# Autodesk Inventor assembly: Lady Brown LS Axle (Left)
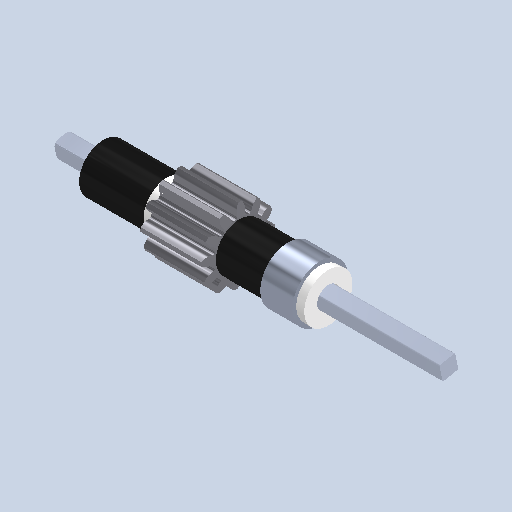
[picture p0: Inventor's stored thumbnail of the model, 512x512]
Saved by Autodesk Inventor 2025.1 (Build 291241020, 241B)
## iProperties
Created: 2024-12-19
Part Number: Lady Brown LS Axle (Left)
Document SubType Name: Assembly
Designer: Juan
Author: Juan
## Documents named in this file (11)
- C:\Users\AtuStem\Documents\GitHub\ATUM-V5RC-High-Stakes-CAD\Robot\Subassemblies\Lady Brown LS Axle (Left).iam
- C:\Users\AtuStem\Documents\GitHub\ATUM-V5RC-High-Stakes-CAD\VEX-CAD-Inventor\Motion\Shaft LS\Shaft LS\Shaft LS 3.0.ipt
- C:\Users\Juan\Documents\GitHub\ATUM-VRC-High-Stakes-CAD\VEX-CAD-Inventor\Motion\Shaft LS\Shaft LS.ipt
- C:\Users\AtuStem\Documents\GitHub\ATUM-V5RC-High-Stakes-CAD\VEX-CAD-Inventor\Motion\Shaft LS\Shaft Collar Metal\Shaft Collar No Screw.ipt
- C:\Users\AtuStem\Documents\GitHub\ATUM-V5RC-High-Stakes-CAD\VEX-CAD-Inventor\Motion\Gears\HS Gear\HS 12T Gear, Square.iam
- C:\Users\Juan\Documents\GitHub\ATUM-VRC-High-Stakes-CAD\VEX-CAD-Inventor\Motion\Gears\HS Gear.iam
- C:\Users\AtuStem\Documents\GitHub\ATUM-V5RC-High-Stakes-CAD\VEX-CAD-Inventor\Motion\Spacers\Spacer Nylon .375 OD\NSpacer .375 OD x .375.ipt
- C:\Users\Juan\Documents\GitHub\ATUM-VRC-High-Stakes-CAD\VEX-CAD-Inventor\Motion\Spacers\Spacer Nylon .375 OD.ipt
- C:\Users\AtuStem\Documents\GitHub\ATUM-V5RC-High-Stakes-CAD\VEX-CAD-Inventor\Motion\Spacers\Washer Teflon\TWasher .375 OD x .06250.ipt
- C:\Users\Juan\Documents\GitHub\ATUM-VRC-High-Stakes-CAD\VEX-CAD-Inventor\Motion\Spacers\Washer Teflon.ipt
- C:\Users\AtuStem\Documents\GitHub\ATUM-V5RC-High-Stakes-CAD\VEX-CAD-Inventor\Motion\Spacers\Spacer Nylon .375 OD\NSpacer .375 OD x .500.ipt
## Components (7 placed, 6 different names)
1. Shaft LS 3.0:1
2. Shaft Collar No Screw:1
3. HS 12T Gear, Square:1 [sub-assembly]
4. NSpacer .375 OD x .375:1
5. TWasher .375 OD x .06250:1
6. TWasher .375 OD x .06250:2
7. NSpacer .375 OD x .500:2
## Relationships (11: Mate 10, Angle 1)
- [Mate]: Shaft LS 3.0:1 ↔ HS 12T Gear, Square:1
- [Mate]: Shaft LS 3.0:1 ↔ HS 12T Gear, Square:1
- [Mate]: Shaft Collar No Screw:1 ↔ NSpacer .375 OD x .375:1
- [Mate]: HS 12T Gear, Square:1 ↔ NSpacer .375 OD x .375:1
- [Mate]: Shaft Collar No Screw:1 ↔ TWasher .375 OD x .06250:1
- [Mate]: HS 12T Gear, Square:1 ↔ TWasher .375 OD x .06250:2
- [Mate]: TWasher .375 OD x .06250:2 ↔ NSpacer .375 OD x .500:2
- [Mate]: TWasher .375 OD x .06250:2 ↔ NSpacer .375 OD x .500:2
- [Mate]: Shaft Collar No Screw:1 ↔ NSpacer .375 OD x .375:1
- [Mate]: NSpacer .375 OD x .375:1 ↔ NSpacer .375 OD x .500:2
- [Angle] (0 deg): Shaft LS 3.0:1 ↔ Shaft Collar No Screw:1
